# Autodesk Inventor assembly: ALPHA FULL
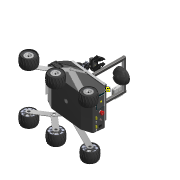
[picture p0: Inventor's stored thumbnail of the model, 180x180]
Saved by Autodesk Inventor 2018 (Build 220112000, 112)
## iProperties
Created: 2014-12-07
Part Number: ALPHA FULL
Document SubType Name: Assembly
Designer: Elev
_SolveAssemblyDoc: Frame Generator Solve Assembly
_Version: 15.0.0
Author: Elev
## Documents named in this file (31)
- C:\Users\cristian\Desktop\correciones y Formato trabajo de grado\ALPHA FULL.iam
- C:\Users\cristian\Desktop\ARCHIVOS 2018-B\AUTODESK INVENTOR\DISEÑO ROVER ALTERNA\ALTERNATIVA5\Rocker Bogie Prototype\Main_leg.ipt
- C:\Users\cristian\Desktop\ARCHIVOS 2018-B\AUTODESK INVENTOR\DISEÑO ROVER ALTERNA\ALTERNATIVA5\Rocker Bogie Prototype\Sub_Leg.ipt
- C:\Users\cristian\Desktop\ARCHIVOS 2018-B\AUTODESK INVENTOR\DISEÑO ROVER ALTERNA\ALTERNATIVA5\Rocker Bogie Prototype\Main_Pipe.ipt
- C:\Users\cristian\Desktop\ARCHIVOS 2018-B\AUTODESK INVENTOR\DISEÑO ROVER ALTERNA\ALTERNATIVA5\Rocker Bogie Prototype\Wheel.ipt
- C:\Users\cristian\Desktop\ARCHIVOS 2018-B\AUTODESK INVENTOR\DISEÑO ROVER ALTERNA\ALTERNATIVA5\Rocker Bogie Prototype\Stabilizer_Connection_Axis.ipt
- C:\Users\cristian\Desktop\ARCHIVOS 2018-B\AUTODESK INVENTOR\DISEÑO ROVER ALTERNA\ALTERNATIVA5\Rocker Bogie Prototype\Main_Body.ipt
- C:\Users\cristian\Desktop\ARCHIVOS 2018-B\AUTODESK INVENTOR\DISEÑO ROVER ALTERNA\ALTERNATIVA5\Rocker Bogie Prototype\Wheel_2.ipt
- C:\Users\cristian\Desktop\ARCHIVOS 2018-B\AUTODESK INVENTOR\DISEÑO ROVER ALTERNA\ALTERNATIVA5\Rocker Bogie Prototype\Body_Side.ipt
- C:\Users\cristian\Desktop\ARCHIVOS 2018-B\AUTODESK INVENTOR\DISEÑO ROVER ALTERNA\ALTERNATIVA5\Rocker Bogie Prototype\Assembly1 SolarUp\Frame\Frame0001.iam
- C:\Users\cristian\Documents\Inventor\DISEÑO ROVER\JAJAJA.iam
- C:\Users\cristian\Documents\Inventor\DISEÑO ROVER\JAJA.iam
- C:\Users\cristian\Documents\Inventor\DISEÑO ROVER\JA.iam
- C:\Users\cristian\Documents\Inventor\DISEÑO ROVER\Part19.ipt
- C:\Users\cristian\Desktop\ARCHIVOS 2018-B\AUTODESK INVENTOR\BOTON EMERGENCIA\Mushroom Emergency PushButton Alon R.ipt
- C:\Users\cristian\Desktop\ARCHIVOS 2018-B\AUTODESK INVENTOR\PANTALLA LCD\Pantalla TFT_320QVT.ipt
- C:\Users\cristian\Desktop\ARCHIVOS 2018-B\AUTODESK INVENTOR\SWITCH\19x13-On-Off-Switch.ipt
- C:\Users\cristian\Desktop\ARCHIVOS 2018-B\AUTODESK INVENTOR\SWITCH\Тумблер PST-121A_IP67.ipt
- C:\Users\cristian\Desktop\ARCHIVOS 2018-B\AUTODESK INVENTOR\CONNECTORE\xt90_female.ipt
- C:\Users\cristian\Desktop\ARCHIVOS 2018-B\AUTODESK INVENTOR\CONNECTORE\User Library-XH2_54-4P-AW.ipt
- C:\Users\cristian\Desktop\ARCHIVOS 2018-B\AUTODESK INVENTOR\CONNECTORE\femaleThruHoleUSB.ipt
- C:\Users\cristian\Desktop\ARCHIVOS 2018-B\AUTODESK INVENTOR\WEBCAM\dome-camera-1.snapshot.3\Âêëàäûø.ipt
- C:\Users\cristian\Desktop\ARCHIVOS 2018-B\AUTODESK INVENTOR\IMU\Mk5 MTi-10 Encased.ipt
- C:\Users\cristian\Desktop\ARCHIVOS 2018-B\AUTODESK INVENTOR\KINECT\AS1.ipt
- C:\Users\cristian\Desktop\ARCHIVOS 2018-B\AUTODESK INVENTOR\DISEÑO ROVER ALTERNA\ALTERNATIVA3\robo wheel.ipt
- C:\Users\cristian\Documents\Inventor\DISEÑO ROVER\JAJAJAJA.iam
- C:\Users\cristian\Documents\Inventor\DISEÑO ROVER\Part57.ipt
- C:\Users\cristian\Documents\Inventor\DISEÑO ROVER\Part64.ipt
- C:\Users\cristian\Desktop\ARCHIVOS 2018-B\AUTODESK INVENTOR\BRAZO\Robotic arm CAD design files\Full assembly.ipt
- C:\Users\cristian\Desktop\ARCHIVOS 2018-B\AUTODESK INVENTOR\TPLINK\Piratebox.ipt
- C:\Users\cristian\Downloads\Led Lens.ipt
## Components (47 placed, 30 different names)
1. Main_leg:1 — Mate:1, Mate:2, Mate:6, Flush:1, Angle:2, Angle:4, Mate:53, Mate:54, Mate:61
2. Sub_Leg:1 — Mate:1, Mate:2, Mate:51, Mate:52, Mate:55
3. Main_leg:2 — Mate:4, Mate:5, Mate:7, Flush:2, Mate:9, Mate:17, Mate:59
4. Sub_Leg:2 — Mate:4, Mate:5, Mate:14, Mate:15, Mate:16
5. Main_Pipe:1 — Mate:6, Mate:7, Flush:1, Flush:2, Mate:58, Mate:60
6. Wheel:4 — Mate:9, Mate:17
7. Wheel:5 — Flush:4, Mate:14, Mate:15
8. Wheel:6 — Flush:4, Mate:16
9. Stabilizer_Connection_Axis:1 — Angle:3, Mate:60, Mate:61, Angle:8
10. Stabilizer_Connection_Axis:2 — Angle:3, Mate:58, Mate:59
11. Main_Body:1 — Angle:2, Angle:4, Angle:8, Mate:89, Mate:90, Flush:7, Flush:8, Mate:91, Mate:92, Flush:11
12. Wheel_2:1 — Mate:53, Mate:54
13. Wheel_2:2 — Mate:52, Flush:5
14. Wheel_2:3 — Mate:51, Flush:5, Mate:55
15. Body_Side:1 — Mate:89, Mate:90, Flush:7
16. Frame0001:1 [sub-assembly] — Flush:10
17. JAJAJA:1 [sub-assembly] — Flush:9
18. JAJA:1 [sub-assembly]
19. JA:1 [sub-assembly]
20. Part19:1 — Flush:9
21. Pantalla TFT_320QVT:1
22. 19x13-On-Off-Switch:2
23. Тумблер PST-121A_IP67:5
24. xt90_female:2
25. xt90_female:3
26. User Library-XH2_54-4P-AW:4
27. User Library-XH2_54-4P-AW:5
28. femaleThruHoleUSB:2
29. femaleThruHoleUSB:3
30. Âêëàäûø:5
31. Mk5 MTi-10 Encased:1
32. AS1:5
33. robo wheel:3
34. robo wheel:4
35. robo wheel:5
36. robo wheel:6
37. robo wheel:7
38. robo wheel:8
39. JAJAJAJA:1 [sub-assembly]
40. Part57:1 — Flush:10
41. Part64:1 — Flush:11
42. Full assembly:1
43. Piratebox:2
44. Led Lens:2
45. Led Lens:3
46. Body_Side:2 — Flush:8, Mate:91, Mate:92
47. Mushroom Emergency PushButton Alon R:2
## Relationships (37: Mate 24, Flush 9, Angle 4)
- Mate:1: Main_leg:1 ↔ Sub_Leg:1
- Mate:2: Main_leg:1 ↔ Sub_Leg:1
- Mate:4: Main_leg:2 ↔ Sub_Leg:2
- Mate:5: Main_leg:2 ↔ Sub_Leg:2
- Mate:6: Main_leg:1 ↔ Main_Pipe:1
- Mate:7: Main_leg:2 ↔ Main_Pipe:1
- Flush:1: Main_leg:1 ↔ Main_Pipe:1
- Flush:2: Main_leg:2 ↔ Main_Pipe:1
- Flush:4: Wheel:5 ↔ Wheel:6
- Mate:9: Main_leg:2 ↔ Wheel:4
- Mate:14: Sub_Leg:2 ↔ Wheel:5
- Mate:15: Sub_Leg:2 ↔ Wheel:5
- Mate:16: Sub_Leg:2 ↔ Wheel:6
- Mate:17: Main_leg:2 ↔ Wheel:4
- Angle:2 (0 deg): Main_leg:1 ↔ Main_Body:1
- Angle:3 (0 deg): Stabilizer_Connection_Axis:1 ↔ Stabilizer_Connection_Axis:2
- Angle:4 (338.2 deg): Main_leg:1 ↔ Main_Body:1
- Mate:51: Sub_Leg:1 ↔ Wheel_2:3
- Mate:52: Sub_Leg:1 ↔ Wheel_2:2
- Mate:53: Main_leg:1 ↔ Wheel_2:1
- Mate:54: Main_leg:1 ↔ Wheel_2:1
- Flush:5: Wheel_2:2 ↔ Wheel_2:3
- Mate:55: Sub_Leg:1 ↔ Wheel_2:3
- Mate:58: Main_Pipe:1 ↔ Stabilizer_Connection_Axis:2
- Mate:59: Main_leg:2 ↔ Stabilizer_Connection_Axis:2
- Mate:60: Main_Pipe:1 ↔ Stabilizer_Connection_Axis:1
- Mate:61: Main_leg:1 ↔ Stabilizer_Connection_Axis:1
- Angle:8 (30 deg): Stabilizer_Connection_Axis:1 ↔ Main_Body:1
- Mate:89: Main_Body:1 ↔ Body_Side:1
- Mate:90: Main_Body:1 ↔ Body_Side:1
- Flush:7 (5 mm): Main_Body:1 ↔ Body_Side:1
- Flush:8 (5 mm): Main_Body:1 ↔ Body_Side:2
- Mate:91: Main_Body:1 ↔ Body_Side:2
- Mate:92: Main_Body:1 ↔ Body_Side:2
- Flush:9: JAJAJA:1 ↔ Part19:1
- Flush:10: Frame0001:1 ↔ Part57:1
- Flush:11: Main_Body:1 ↔ Part64:1
